# Autodesk Inventor assembly: Assembly1
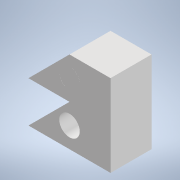
[picture p0: Inventor's stored thumbnail of the model, 180x180]
Saved by Autodesk Inventor 2020 (Build 240168000, 168)
## iProperties
Created: 2021-04-22
Part Number: Assembly1
Document SubType Name: Assembly
Designer: adriggs
Author: adriggs
## Documents named in this file (3)
- I:\3D Modeling\Assembly\Assembly1.iam
- I:\3D Modeling\Assembly\block.ipt
- I:\3D Modeling\Assembly\cylinder.ipt
## Components (3 placed, 2 different names)
1. block:1 — Mate:1, Mate:2, Flush:1
2. block:2 — Mate:1, Mate:2, Flush:1
3. cylinder:1
## Relationships (3: Mate 2, Flush 1)
- Mate:1: block:1 ↔ block:2
- Mate:2: block:1 ↔ block:2
- Flush:1: block:1 ↔ block:2
